# Autodesk Inventor assembly: Baugruppe1
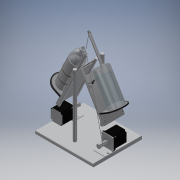
[picture p0: Inventor's stored thumbnail of the model, 180x180]
Saved by Autodesk Inventor 2019 (Build 230136000, 136)
## iProperties
Created: 2018-11-28
Part Number: Baugruppe1
Material: Generisch
Document SubType Name: Assembly
Designer: nico-
Author: nico-
## Documents named in this file (21)
- C:\Users\nico-\Dropbox\GEM CAD\Baugruppe 1\Baugruppe1.iam
- C:\Users\nico-\Dropbox\GEM CAD\Einzelteile Antrieb\Bodenplatte.ipt
- C:\Users\nico-\Dropbox\GEM CAD\Einzelteile Antrieb\Hauptpfeiler.ipt
- C:\Users\nico-\Dropbox\GEM CAD\Einzelteile Antrieb\Drehstange.ipt
- C:\Users\nico-\Dropbox\GEM CAD\Einzelteile Antrieb\Stange FlascheGlas kurz.ipt
- C:\Users\nico-\Dropbox\GEM CAD\Einzelteile Antrieb\Stange FlascheGlas.ipt
- C:\Users\nico-\Dropbox\GEM CAD\Einzelteile Antrieb\Halterungshauptplatte.ipt
- C:\Users\nico-\Dropbox\GEM CAD\Einzelteile Antrieb\Flasche.ipt
- C:\Users\nico-\Dropbox\GEM CAD\Einzelteile Antrieb\Motor.ipt
- C:\Users\nico-\Dropbox\GEM CAD\Einzelteile Antrieb\Motorhalterung.ipt
- C:\Users\nico-\Dropbox\GEM CAD\Einzelteile Antrieb\Glas und Flaschenboden.ipt
- C:\Users\nico-\Dropbox\GEM CAD\Einzelteile Antrieb\Glashalter.ipt
- C:\Users\nico-\Dropbox\GEM CAD\Einzelteile Antrieb\Glas.ipt
- C:\Users\nico-\Dropbox\GEM CAD\Einzelteile Antrieb\Wasser.ipt
- C:\Users\nico-\Dropbox\GEM CAD\Einzelteile Antrieb\Flaschenetikette.ipt
- C:\Users\nico-\Dropbox\GEM CAD\Einzelteile Antrieb\Flaschenhalter.ipt
- C:\Users\nico-\Dropbox\GEM CAD\Einzelteile Antrieb\Seil.ipt
- C:\Users\nico-\Documents\Inventor\Content Center Files\R2019\de-DE\ISO 4762(1)\DIN EN ISO 4762 - M6 x 10.ipt
- C:\Users\nico-\Documents\Inventor\Content Center Files\R2019\de-DE\ISO 4017(1)\ISO 4017 - M5 x 10 - ISO.ipt
- C:\Users\nico-\Documents\Inventor\Content Center Files\R2019\de-DE\DIN 7985 (Z)\DIN 7985 (Z) - M5x16-Z.ipt
- C:\Users\nico-\Documents\Inventor\Content Center Files\R2019\de-DE\DIN 7985 (Z)\DIN 7985 (Z) - M4x16-Z.ipt
## Components (40 placed, 20 different names)
1. Bodenplatte:1 — Passend:1, Passend:2, Fluchtend:1, Passend:3, Passend:4, Passend:19, Passend:23, Passend:28, Fluchtend:5, Fluchtend:6, Passend:30, Passend:33, Passend:35, Passend:36, Passend:41
2. Hauptpfeiler:1 — Passend:3, Passend:7, Fluchtend:3, Passend:19, Passend:22
3. Hauptpfeiler:2 — Passend:4, Passend:8, Fluchtend:2, Passend:21, Passend:23
4. Drehstange:1 — Passend:12, Passend:13, Passend:14, Passend:21, Passend:22, Passend:24
5. Stange FlascheGlas kurz:1 — Passend:16, Tangential:1, Passend:24
6. Stange FlascheGlas kurz:2 — Passend:12, Passend:17
7. Stange FlascheGlas:1 — Passend:13, Passend:18, Tangential:2, Fluchtend:2, Passend:53
8. Stange FlascheGlas:2 — Passend:14, Passend:15, Fluchtend:3, Passend:52
9. Halterungshauptplatte:1 — Passend:15, Passend:16, Tangential:1, Passend:25, Passend:26, Passend:37, Fluchtend:8, Passend:38
10. Halterungshauptplatte:2 — Passend:17, Passend:18, Tangential:2, Passend:40, Fluchtend:9, Fluchtend:10, Passend:42, Fluchtend:11, Passend:43, Passend:45, Passend:54, Passend:56
11. Flasche:1 — Passend:25, Passend:26, Passend:39, Passend:49, Passend:50
12. Motor:1 — Fluchtend:6, Passend:30, Passend:32, Fluchtend:7
13. Motor:2 — Passend:28, Fluchtend:5, Passend:34
14. Motorhalterung:1 — Passend:34, Passend:35, Passend:36, Passend:41, Passend:60, Passend:61, Passend:62, Passend:63, Passend:64, Passend:65, Passend:66, Passend:67, Passend:68, Passend:69, Passend:70
15. Motorhalterung:2 — Passend:32, Passend:33, Fluchtend:7, Passend:71, Passend:72, Passend:73, Passend:74, Passend:75, Passend:76, Passend:77, Passend:78
16. Glas und Flaschenboden:1 — Passend:40, Fluchtend:9, Fluchtend:10, Passend:44, Passend:46, Passend:55
17. Glas und Flaschenboden:2 — Passend:37, Fluchtend:8, Passend:38, Passend:39, Passend:51
18. Glashalter:1 — Passend:42, Fluchtend:11, Passend:43, Passend:57, Passend:58, Passend:59
19. Glas:1 — Passend:44, Passend:45, Passend:46, Passend:47, Passend:48
20. Wasser:1 — Passend:47, Passend:48
21. Flaschenetikette:1 — Passend:49
22. Flaschenhalter:1 — Passend:50, Passend:51
23. Seil:1
24. Seil:2
25. DIN EN ISO 4762 M6 x 10:1 — Passend:52
26. DIN EN ISO 4762 M6 x 10:2 — Passend:53
27. ISO 4017 M5 x 10:1 — Passend:54, Passend:55
28. ISO 4017 M5 x 10:2 — Passend:56
29. ISO 4017 M5 x 10:3 — Passend:58
30. ISO 4017 M5 x 10:4 — Passend:57, Passend:59
31. ISO 4017 M5 x 10:5 — Passend:60, Passend:61
32. ISO 4017 M5 x 10:6 — Passend:62
33. DIN 7985 (Z) M5x16-Z:1 — Passend:63, Passend:67
34. DIN 7985 (Z) M5x16-Z:2 — Passend:66, Passend:68
35. DIN 7985 (Z) M5x16-Z:3 — Passend:65, Passend:70
36. DIN 7985 (Z) M5x16-Z:4 — Passend:64, Passend:69
37. DIN 7985 (Z) M4x16-Z:1 — Passend:73, Passend:77
38. DIN 7985 (Z) M4x16-Z:2 — Passend:74, Passend:78
39. DIN 7985 (Z) M4x16-Z:3 — Passend:72, Passend:75
40. DIN 7985 (Z) M4x16-Z:4 — Passend:71, Passend:76
## Relationships (81: Mate 69, Flush 10, Tangent 2)
- Passend:1 [Mate]: Bodenplatte:1
- Passend:2 [Mate] (-125 mm): Bodenplatte:1
- Fluchtend:1 [Flush] (-175 mm): Bodenplatte:1
- Passend:3 [Mate]: Bodenplatte:1 ↔ Hauptpfeiler:1
- Passend:4 [Mate]: Bodenplatte:1 ↔ Hauptpfeiler:2
- Passend:7 [Mate]: Hauptpfeiler:1
- Passend:8 [Mate]: Hauptpfeiler:2
- Passend:12 [Mate] (1 mm): Drehstange:1 ↔ Stange FlascheGlas kurz:2
- Passend:13 [Mate]: Drehstange:1 ↔ Stange FlascheGlas:1
- Passend:14 [Mate]: Drehstange:1 ↔ Stange FlascheGlas:2
- Passend:15 [Mate]: Stange FlascheGlas:2 ↔ Halterungshauptplatte:1
- Passend:16 [Mate]: Stange FlascheGlas kurz:1 ↔ Halterungshauptplatte:1
- Tangential:1: Stange FlascheGlas kurz:1 ↔ Halterungshauptplatte:1
- Passend:17 [Mate]: Stange FlascheGlas kurz:2 ↔ Halterungshauptplatte:2
- Passend:18 [Mate]: Stange FlascheGlas:1 ↔ Halterungshauptplatte:2
- Tangential:2 (3 mm): Stange FlascheGlas:1 ↔ Halterungshauptplatte:2
- Fluchtend:2 [Flush] (16.5 mm): Hauptpfeiler:2 ↔ Stange FlascheGlas:1
- Fluchtend:3 [Flush] (15.5 mm): Hauptpfeiler:1 ↔ Stange FlascheGlas:2
- Passend:19 [Mate]: Bodenplatte:1 ↔ Hauptpfeiler:1
- Passend:21 [Mate]: Hauptpfeiler:2 ↔ Drehstange:1
- Passend:22 [Mate] (-8 mm): Hauptpfeiler:1 ↔ Drehstange:1
- Passend:23 [Mate]: Bodenplatte:1 ↔ Hauptpfeiler:2
- Passend:24 [Mate]: Drehstange:1 ↔ Stange FlascheGlas kurz:1
- Passend:25 [Mate] (35 mm): Halterungshauptplatte:1 ↔ Flasche:1
- Passend:26 [Mate] (-50 mm): Halterungshauptplatte:1 ↔ Flasche:1
- Passend:28 [Mate] (5 mm): Bodenplatte:1 ↔ Motor:2
- Fluchtend:5 [Flush] (105 mm): Bodenplatte:1 ↔ Motor:2
- Fluchtend:6 [Flush] (105 mm): Bodenplatte:1 ↔ Motor:1
- Passend:30 [Mate] (5 mm): Bodenplatte:1 ↔ Motor:1
- Passend:32 [Mate]: Motor:1 ↔ Motorhalterung:2
- Passend:33 [Mate]: Bodenplatte:1 ↔ Motorhalterung:2
- Fluchtend:7 [Flush]: Motor:1 ↔ Motorhalterung:2
- Passend:34 [Mate]: Motor:2 ↔ Motorhalterung:1
- Passend:35 [Mate]: Bodenplatte:1 ↔ Motorhalterung:1
- Passend:36 [Mate]: Bodenplatte:1 ↔ Motorhalterung:1
- Passend:37 [Mate]: Halterungshauptplatte:1 ↔ Glas und Flaschenboden:2
- Fluchtend:8 [Flush] (-1 mm): Halterungshauptplatte:1 ↔ Glas und Flaschenboden:2
- Passend:38 [Mate]: Halterungshauptplatte:1 ↔ Glas und Flaschenboden:2
- Passend:39 [Mate]: Flasche:1 ↔ Glas und Flaschenboden:2
- Passend:40 [Mate]: Halterungshauptplatte:2 ↔ Glas und Flaschenboden:1
- Fluchtend:9 [Flush] (-1 mm): Halterungshauptplatte:2 ↔ Glas und Flaschenboden:1
- Fluchtend:10 [Flush]: Halterungshauptplatte:2 ↔ Glas und Flaschenboden:1
- Passend:41 [Mate]: Bodenplatte:1 ↔ Motorhalterung:1
- Passend:42 [Mate]: Halterungshauptplatte:2 ↔ Glashalter:1
- Fluchtend:11 [Flush]: Halterungshauptplatte:2 ↔ Glashalter:1
- Passend:43 [Mate]: Halterungshauptplatte:2 ↔ Glashalter:1
- Passend:44 [Mate]: Glas und Flaschenboden:1 ↔ Glas:1
- Passend:45 [Mate] (-51 mm): Halterungshauptplatte:2 ↔ Glas:1
- Passend:46 [Mate] (39 mm): Glas und Flaschenboden:1 ↔ Glas:1
- Passend:47 [Mate]: Glas:1 ↔ Wasser:1
- Passend:48 [Mate]: Glas:1 ↔ Wasser:1
- Passend:49 [Mate]: Flasche:1 ↔ Flaschenetikette:1
- Passend:50 [Mate]: Flasche:1 ↔ Flaschenhalter:1
- Passend:51 [Mate]: Glas und Flaschenboden:2 ↔ Flaschenhalter:1
- Passend:52 [Mate]: Stange FlascheGlas:2 ↔ DIN EN ISO 4762 M6 x 10:1
- Passend:53 [Mate]: Stange FlascheGlas:1 ↔ DIN EN ISO 4762 M6 x 10:2
- Passend:54 [Mate]: Halterungshauptplatte:2 ↔ ISO 4017 M5 x 10:1
- Passend:55 [Mate]: Glas und Flaschenboden:1 ↔ ISO 4017 M5 x 10:1
- Passend:56 [Mate]: Halterungshauptplatte:2 ↔ ISO 4017 M5 x 10:2
- Passend:57 [Mate]: Glashalter:1 ↔ ISO 4017 M5 x 10:4
- Passend:58 [Mate]: Glashalter:1 ↔ ISO 4017 M5 x 10:3
- Passend:59 [Mate]: Glashalter:1 ↔ ISO 4017 M5 x 10:4
- Passend:60 [Mate]: Motorhalterung:1 ↔ ISO 4017 M5 x 10:5
- Passend:61 [Mate]: Motorhalterung:1 ↔ ISO 4017 M5 x 10:5
- Passend:62 [Mate]: Motorhalterung:1 ↔ ISO 4017 M5 x 10:6
- Passend:63 [Mate]: Motorhalterung:1 ↔ DIN 7985 (Z) M5x16-Z:1
- Passend:64 [Mate]: Motorhalterung:1 ↔ DIN 7985 (Z) M5x16-Z:4
- Passend:65 [Mate]: Motorhalterung:1 ↔ DIN 7985 (Z) M5x16-Z:3
- Passend:66 [Mate]: Motorhalterung:1 ↔ DIN 7985 (Z) M5x16-Z:2
- Passend:67 [Mate]: Motorhalterung:1 ↔ DIN 7985 (Z) M5x16-Z:1
- Passend:68 [Mate]: Motorhalterung:1 ↔ DIN 7985 (Z) M5x16-Z:2
- Passend:69 [Mate]: Motorhalterung:1 ↔ DIN 7985 (Z) M5x16-Z:4
- Passend:70 [Mate]: Motorhalterung:1 ↔ DIN 7985 (Z) M5x16-Z:3
- Passend:71 [Mate]: Motorhalterung:2 ↔ DIN 7985 (Z) M4x16-Z:4
- Passend:72 [Mate]: Motorhalterung:2 ↔ DIN 7985 (Z) M4x16-Z:3
- Passend:73 [Mate]: Motorhalterung:2 ↔ DIN 7985 (Z) M4x16-Z:1
- Passend:74 [Mate]: Motorhalterung:2 ↔ DIN 7985 (Z) M4x16-Z:2
- Passend:75 [Mate]: Motorhalterung:2 ↔ DIN 7985 (Z) M4x16-Z:3
- Passend:76 [Mate]: Motorhalterung:2 ↔ DIN 7985 (Z) M4x16-Z:4
- Passend:77 [Mate]: Motorhalterung:2 ↔ DIN 7985 (Z) M4x16-Z:1
- Passend:78 [Mate]: Motorhalterung:2 ↔ DIN 7985 (Z) M4x16-Z:2
